# Autodesk Inventor assembly: Assembly1
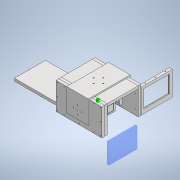
[picture p0: Inventor's stored thumbnail of the model, 180x180]
Saved by Autodesk Inventor 2022.2 (Build 262287030, 287C)
## iProperties
Created: 2022-01-28
Part Number: Assembly1
Document SubType Name: Assembly
Designer: Tapendra
Author: Tapendra
## Documents named in this file (25)
- C:\Users\Tapendra\Documents\opticalbox\Assembly1.iam
- C:\Users\Tapendra\Documents\opticalbox\base.ipt
- C:\Users\Tapendra\Documents\opticalbox\back.ipt
- C:\Users\Tapendra\Documents\opticalbox\top.ipt
- C:\Users\Tapendra\Documents\opticalbox\leftright.ipt
- C:\Users\Tapendra\Documents\opticalbox\CCM1-BS013.ipt
- C:\Users\Tapendra\Documents\opticalbox\front.ipt
- C:\Users\Tapendra\Documents\opticalbox\topwindow.ipt
- C:\Users\Tapendra\Documents\opticalbox\acrylicpmt.ipt
- C:\Users\Tapendra\Documents\opticalbox\toppmt.ipt
- C:\Users\Tapendra\Documents\opticalbox\left.ipt
- C:\Users\Tapendra\Documents\opticalbox\SM1D12-Step.ipt
- C:\Users\Tapendra\Documents\opticalbox\ELL14K-Step.ipt
- C:\Users\Tapendra\Documents\opticalbox\CFC11P-A-Step.ipt
- C:\Users\Tapendra\Documents\opticalbox\WP25M-UB-Step.ipt
- C:\Users\Tapendra\Documents\opticalbox\92078A216_Polycarbonate Dowel Pin.ipt
- C:\Users\Tapendra\Documents\opticalbox\baseblock.ipt
- C:\Users\Tapendra\Documents\opticalbox\baseplate.ipt
- C:\Users\Tapendra\Documents\opticalbox\MOT1102_0_3D.iam
- C:\Users\Tapendra\Documents\opticalbox\94180A351_Tapered Heat-Set Inserts for Plastic.ipt
- C:\Users\Tapendra\Documents\opticalbox\sidebracket.ipt
- C:\Users\Tapendra\Documents\opticalbox\pmtholder.ipt
- C:\Users\Tapendra\Documents\opticalbox\pmtbase.ipt
- C:\Users\Tapendra\Documents\Inventor\Content Center Files\R2022\en-US\UNI EN ISO 7045  H\EN ISO 7045 - M2 x  6 - 4.8 - H.ipt
- C:\Users\Tapendra\Documents\opticalbox\acrylicwindow.ipt
## Components (76 placed, 24 different names)
1. base:1 — Mate:1, Flush:1, Flush:2, Flush:8, Flush:9, Mate:15, Mate:24, Mate:25, Mate:26, Mate:27, Mate:33, Mate:34, Mate:35, Mate:57, Mate:60, Mate:61, Mate:64, Mate:86, Mate:92, Mate:131, Mate:132, Mate:133, Mate:134, Mate:135, Mate:136, Mate:137, Mate:138, Mate:144, Mate:145, Mate:146, Mate:147, Mate:148, Mate:149, Mate:150, Mate:151, Mate:153, Mate:154
2. back:1 — Mate:1, Flush:1, Flush:2, Mate:2, Flush:3, Flush:4, Mate:7, Mate:13, Mate:36, Mate:37, Mate:38, Mate:39, Mate:50, Mate:51, Mate:55, Mate:56, Mate:66, Mate:68, Mate:81, Mate:82, Mate:83, Mate:84, Mate:125, Mate:126, Mate:141, Mate:142
3. top:1 — Mate:2, Flush:3, Flush:4, Mate:5, Flush:6, Mate:6, Flush:7, Mate:73, Mate:74, Mate:75, Mate:76, Mate:77, Mate:78, Mate:79, Mate:80, Mate:94, Mate:95, Mate:96, Mate:97, Mate:98, Mate:99, Mate:100, Mate:101, Mate:102, Mate:103, Mate:104, Mate:105, Mate:106, Mate:107, Mate:108, Mate:109, Mate:110, Mate:111, Mate:112, Mate:113, Mate:114, Mate:115, Mate:116, Mate:117
4. front:1 — Mate:5, Flush:6, Mate:40, Mate:41, Mate:42, Mate:43, Mate:44, Mate:45, Mate:46, Mate:47, Mate:48, Mate:52, Mate:53, Mate:54, Mate:69, Mate:70, Mate:71, Mate:72, Mate:143
5. topwindow:1 — Mate:6, Flush:7, Mate:127, Mate:128, Mate:129, Mate:130
6. acrylicpmt:1 — Mate:85
7. leftright:1 — Mate:7, Flush:8, Mate:85
8. toppmt:1 — Mate:139, Mate:140
9. left:1 — Mate:13, Flush:9, Mate:86, Mate:143
10. CFC11P-A-Step:1 — Mate:30
11. ELL14K-Step:1 — Insert:1, Mate:22, Mate:23, Mate:30
12. WP25M-UB-Step:1 — Insert:1
13. CCM1-BS013:2 — Mate:17, Mate:18, Mate:22, Mate:23, Mate:87, Mate:88, Mate:122, Mate:152
14. 92078A216_Polycarbonate Dowel Pin:1 — Mate:40, Mate:41
15. 92078A216_Polycarbonate Dowel Pin:2 — Mate:26, Mate:27
16. 92078A216_Polycarbonate Dowel Pin:3 — Mate:15, Mate:33
17. 92078A216_Polycarbonate Dowel Pin:4 — Mate:144, Mate:145
18. 92078A216_Polycarbonate Dowel Pin:5 — Mate:34, Mate:35
19. 92078A216_Polycarbonate Dowel Pin:6 — Mate:146, Mate:147
20. 92078A216_Polycarbonate Dowel Pin:7 — Mate:24, Mate:25
21. 92078A216_Polycarbonate Dowel Pin:8 — Mate:38, Mate:39
22. 92078A216_Polycarbonate Dowel Pin:9 — Mate:36, Mate:37
23. SM1D12-Step:1 — Mate:17, Mate:18, Mate:121
24. 92078A216_Polycarbonate Dowel Pin:10 — Mate:53, Mate:54
25. 92078A216_Polycarbonate Dowel Pin:12 — Mate:60, Mate:61
26. 92078A216_Polycarbonate Dowel Pin:13 — Mate:42, Mate:43
27. 92078A216_Polycarbonate Dowel Pin:14 — Mate:50, Mate:56
28. 92078A216_Polycarbonate Dowel Pin:15 — Mate:44, Mate:45
29. 92078A216_Polycarbonate Dowel Pin:16 — Mate:46, Mate:47
30. 92078A216_Polycarbonate Dowel Pin:17 — Mate:48, Mate:52
31. 92078A216_Polycarbonate Dowel Pin:18 — Mate:148, Mate:149
32. 92078A216_Polycarbonate Dowel Pin:19 — Mate:57, Mate:64
33. 92078A216_Polycarbonate Dowel Pin:20 — Mate:150, Mate:151
34. 92078A216_Polycarbonate Dowel Pin:21 — Mate:141, Mate:142
35. 92078A216_Polycarbonate Dowel Pin:22 — Mate:66, Mate:68
36. 92078A216_Polycarbonate Dowel Pin:25 — Mate:51, Mate:55
37. 92078A216_Polycarbonate Dowel Pin:26 — Mate:75, Mate:77
38. 92078A216_Polycarbonate Dowel Pin:27 — Mate:70, Mate:71
39. 92078A216_Polycarbonate Dowel Pin:28 — Mate:74, Mate:79
40. 92078A216_Polycarbonate Dowel Pin:29 — Mate:76, Mate:78
41. 92078A216_Polycarbonate Dowel Pin:30 — Mate:73, Mate:80
42. 92078A216_Polycarbonate Dowel Pin:31 — Mate:81, Mate:82
43. 92078A216_Polycarbonate Dowel Pin:32 — Mate:69, Mate:72
44. 92078A216_Polycarbonate Dowel Pin:36 — Mate:83, Mate:84
45. baseblock:1 — Flush:91, Mate:90, Mate:91, Mate:92, Mate:153, Mate:154
46. baseplate:1 — Mate:87, Mate:88, Mate:89, Mate:91
47. 92078A216_Polycarbonate Dowel Pin:37 — Mate:89, Flush:91, Mate:90
48. MOT1102_0_3D:1 [sub-assembly]
49. 94180A351_Tapered Heat-Set Inserts for Plastic:1 — Mate:134, Mate:135
50. 94180A351_Tapered Heat-Set Inserts for Plastic:2 — Mate:96, Mate:107
51. 94180A351_Tapered Heat-Set Inserts for Plastic:3 — Mate:100, Mate:109
52. 94180A351_Tapered Heat-Set Inserts for Plastic:4 — Mate:102, Mate:111
53. 94180A351_Tapered Heat-Set Inserts for Plastic:5 — Mate:130
54. 94180A351_Tapered Heat-Set Inserts for Plastic:6 — Mate:106, Mate:115
55. 94180A351_Tapered Heat-Set Inserts for Plastic:7 — Mate:99, Mate:116
56. 94180A351_Tapered Heat-Set Inserts for Plastic:8 — Mate:101, Mate:110
57. 94180A351_Tapered Heat-Set Inserts for Plastic:9 — Mate:94, Mate:95
58. 94180A351_Tapered Heat-Set Inserts for Plastic:10 — Mate:97, Mate:108
59. 94180A351_Tapered Heat-Set Inserts for Plastic:11 — Mate:127
60. 94180A351_Tapered Heat-Set Inserts for Plastic:12 — Mate:131, Mate:132
61. 94180A351_Tapered Heat-Set Inserts for Plastic:13 — Mate:98, Mate:117
62. 94180A351_Tapered Heat-Set Inserts for Plastic:14 — Mate:129
63. 94180A351_Tapered Heat-Set Inserts for Plastic:15 — Mate:104, Mate:113
64. 94180A351_Tapered Heat-Set Inserts for Plastic:16 — Mate:105, Mate:114
65. 94180A351_Tapered Heat-Set Inserts for Plastic:17 — Mate:133, Mate:136
66. 94180A351_Tapered Heat-Set Inserts for Plastic:18 — Mate:128
67. 94180A351_Tapered Heat-Set Inserts for Plastic:19 — Mate:103, Mate:112
68. sidebracket:1 — Mate:125, Mate:126
69. pmtholder:1 — Mate:123, Mate:124
70. pmtbase:1 — Mate:121, Mate:122, Mate:123, Mate:124, Mate:139, Mate:140, Mate:152, Insert:3, Mate:155, Insert:4, Mate:156
71. 94180A351_Tapered Heat-Set Inserts for Plastic:20 — Mate:137, Mate:138
72. UNI EN ISO 7045 H M2 x  6 - 4.8 - H:1 — Mate:155
73. UNI EN ISO 7045 H M2 x  6 - 4.8 - H:2 — Mate:156
74. UNI EN ISO 7045 H M2 x  6 - 4.8 - H:3 — Insert:4
75. UNI EN ISO 7045 H M2 x  6 - 4.8 - H:4 — Insert:3
76. acrylicwindow:1
## Relationships (141: Mate 129, Flush 9, Insert 3)
- Mate:1: base:1 ↔ back:1
- Flush:1: base:1 ↔ back:1
- Flush:2: base:1 ↔ back:1
- Mate:2: back:1 ↔ top:1
- Flush:3: back:1 ↔ top:1
- Flush:4: back:1 ↔ top:1
- Mate:5: top:1 ↔ front:1
- Flush:6: top:1 ↔ front:1
- Mate:6: top:1 ↔ topwindow:1
- Flush:7: top:1 ↔ topwindow:1
- Mate:7: back:1 ↔ leftright:1
- Flush:8: base:1 ↔ leftright:1
- Mate:13: back:1 ↔ left:1
- Flush:9: base:1 ↔ left:1
- Insert:1 (-10 mm): ELL14K-Step:1 ↔ WP25M-UB-Step:1
- Mate:15: base:1 ↔ 92078A216_Polycarbonate Dowel Pin:3
- Mate:17: CCM1-BS013:2 ↔ SM1D12-Step:1
- Mate:18: CCM1-BS013:2 ↔ SM1D12-Step:1
- Mate:22: ELL14K-Step:1 ↔ CCM1-BS013:2
- Mate:23: ELL14K-Step:1 ↔ CCM1-BS013:2
- Mate:24: base:1 ↔ 92078A216_Polycarbonate Dowel Pin:7
- Mate:25: base:1 ↔ 92078A216_Polycarbonate Dowel Pin:7
- Mate:26: base:1 ↔ 92078A216_Polycarbonate Dowel Pin:2
- Mate:27: base:1 ↔ 92078A216_Polycarbonate Dowel Pin:2
- Mate:30: CFC11P-A-Step:1 ↔ ELL14K-Step:1
- Mate:33: base:1 ↔ 92078A216_Polycarbonate Dowel Pin:3
- Mate:34: base:1 ↔ 92078A216_Polycarbonate Dowel Pin:5
- Mate:35: base:1 ↔ 92078A216_Polycarbonate Dowel Pin:5
- Mate:36: back:1 ↔ 92078A216_Polycarbonate Dowel Pin:9
- Mate:37: back:1 ↔ 92078A216_Polycarbonate Dowel Pin:9
- Mate:38: back:1 ↔ 92078A216_Polycarbonate Dowel Pin:8
- Mate:39: back:1 ↔ 92078A216_Polycarbonate Dowel Pin:8
- Mate:40: front:1 ↔ 92078A216_Polycarbonate Dowel Pin:1
- Mate:41: front:1 ↔ 92078A216_Polycarbonate Dowel Pin:1
- Mate:42: front:1 ↔ 92078A216_Polycarbonate Dowel Pin:13
- Mate:43: front:1 ↔ 92078A216_Polycarbonate Dowel Pin:13
- Mate:44: front:1 ↔ 92078A216_Polycarbonate Dowel Pin:15
- Mate:45: front:1 ↔ 92078A216_Polycarbonate Dowel Pin:15
- Mate:46: front:1 ↔ 92078A216_Polycarbonate Dowel Pin:16
- Mate:47: front:1 ↔ 92078A216_Polycarbonate Dowel Pin:16
- Mate:48: front:1 ↔ 92078A216_Polycarbonate Dowel Pin:17
- Mate:50: back:1 ↔ 92078A216_Polycarbonate Dowel Pin:14
- Mate:51: back:1 ↔ 92078A216_Polycarbonate Dowel Pin:25
- Mate:52: front:1 ↔ 92078A216_Polycarbonate Dowel Pin:17
- Mate:53: front:1 ↔ 92078A216_Polycarbonate Dowel Pin:10
- Mate:54: front:1 ↔ 92078A216_Polycarbonate Dowel Pin:10
- Mate:55: back:1 ↔ 92078A216_Polycarbonate Dowel Pin:25
- Mate:56: back:1 ↔ 92078A216_Polycarbonate Dowel Pin:14
- Mate:57: base:1 ↔ 92078A216_Polycarbonate Dowel Pin:19
- Mate:60: base:1 ↔ 92078A216_Polycarbonate Dowel Pin:12
- Mate:61: base:1 ↔ 92078A216_Polycarbonate Dowel Pin:12
- Mate:64: base:1 ↔ 92078A216_Polycarbonate Dowel Pin:19
- Mate:66: back:1 ↔ 92078A216_Polycarbonate Dowel Pin:22
- Mate:68: back:1 ↔ 92078A216_Polycarbonate Dowel Pin:22
- Mate:69: front:1 ↔ 92078A216_Polycarbonate Dowel Pin:32
- Mate:70: front:1 ↔ 92078A216_Polycarbonate Dowel Pin:27
- Mate:71: front:1 ↔ 92078A216_Polycarbonate Dowel Pin:27
- Mate:72: front:1 ↔ 92078A216_Polycarbonate Dowel Pin:32
- Mate:73: top:1 ↔ 92078A216_Polycarbonate Dowel Pin:30
- Mate:74: top:1 ↔ 92078A216_Polycarbonate Dowel Pin:28
- Mate:75: top:1 ↔ 92078A216_Polycarbonate Dowel Pin:26
- Mate:76: top:1 ↔ 92078A216_Polycarbonate Dowel Pin:29
- Mate:77: top:1 ↔ 92078A216_Polycarbonate Dowel Pin:26
- Mate:78: top:1 ↔ 92078A216_Polycarbonate Dowel Pin:29
- Mate:79: top:1 ↔ 92078A216_Polycarbonate Dowel Pin:28
- Mate:80: top:1 ↔ 92078A216_Polycarbonate Dowel Pin:30
- Mate:81: back:1 ↔ 92078A216_Polycarbonate Dowel Pin:31
- Mate:82: back:1 ↔ 92078A216_Polycarbonate Dowel Pin:31
- Mate:83: back:1 ↔ 92078A216_Polycarbonate Dowel Pin:36
- Mate:84: back:1 ↔ 92078A216_Polycarbonate Dowel Pin:36
- Mate:85: acrylicpmt:1 ↔ leftright:1
- Mate:86: base:1 ↔ left:1
- Mate:87: CCM1-BS013:2 ↔ baseplate:1
- Mate:88: CCM1-BS013:2 ↔ baseplate:1
- Mate:89: baseplate:1 ↔ 92078A216_Polycarbonate Dowel Pin:37
- Flush:91: baseblock:1 ↔ 92078A216_Polycarbonate Dowel Pin:37
- Mate:90: baseblock:1 ↔ 92078A216_Polycarbonate Dowel Pin:37
- Mate:91: baseblock:1 ↔ baseplate:1
- Mate:92: base:1 ↔ baseblock:1
- Mate:94: top:1 ↔ 94180A351_Tapered Heat-Set Inserts for Plastic:9
- Mate:95: top:1 ↔ 94180A351_Tapered Heat-Set Inserts for Plastic:9
- Mate:96: top:1 ↔ 94180A351_Tapered Heat-Set Inserts for Plastic:2
- Mate:97: top:1 ↔ 94180A351_Tapered Heat-Set Inserts for Plastic:10
- Mate:98: top:1 ↔ 94180A351_Tapered Heat-Set Inserts for Plastic:13
- Mate:99: top:1 ↔ 94180A351_Tapered Heat-Set Inserts for Plastic:7
- Mate:100: top:1 ↔ 94180A351_Tapered Heat-Set Inserts for Plastic:3
- Mate:101: top:1 ↔ 94180A351_Tapered Heat-Set Inserts for Plastic:8
- Mate:102: top:1 ↔ 94180A351_Tapered Heat-Set Inserts for Plastic:4
- Mate:103: top:1 ↔ 94180A351_Tapered Heat-Set Inserts for Plastic:19
- Mate:104: top:1 ↔ 94180A351_Tapered Heat-Set Inserts for Plastic:15
- Mate:105: top:1 ↔ 94180A351_Tapered Heat-Set Inserts for Plastic:16
- Mate:106: top:1 ↔ 94180A351_Tapered Heat-Set Inserts for Plastic:6
- Mate:107: top:1 ↔ 94180A351_Tapered Heat-Set Inserts for Plastic:2
- Mate:108: top:1 ↔ 94180A351_Tapered Heat-Set Inserts for Plastic:10
- Mate:109: top:1 ↔ 94180A351_Tapered Heat-Set Inserts for Plastic:3
- Mate:110: top:1 ↔ 94180A351_Tapered Heat-Set Inserts for Plastic:8
- Mate:111: top:1 ↔ 94180A351_Tapered Heat-Set Inserts for Plastic:4
- Mate:112: top:1 ↔ 94180A351_Tapered Heat-Set Inserts for Plastic:19
- Mate:113: top:1 ↔ 94180A351_Tapered Heat-Set Inserts for Plastic:15
- Mate:114: top:1 ↔ 94180A351_Tapered Heat-Set Inserts for Plastic:16
- Mate:115: top:1 ↔ 94180A351_Tapered Heat-Set Inserts for Plastic:6
- Mate:116: top:1 ↔ 94180A351_Tapered Heat-Set Inserts for Plastic:7
- Mate:117: top:1 ↔ 94180A351_Tapered Heat-Set Inserts for Plastic:13
- Mate:121: SM1D12-Step:1 ↔ pmtbase:1
- Mate:122: CCM1-BS013:2 ↔ pmtbase:1
- Mate:123: pmtholder:1 ↔ pmtbase:1
- Mate:124: pmtholder:1 ↔ pmtbase:1
- Mate:125: back:1 ↔ sidebracket:1
- Mate:126 (20 mm): back:1 ↔ sidebracket:1
- Mate:127: topwindow:1 ↔ 94180A351_Tapered Heat-Set Inserts for Plastic:11
- Mate:128: topwindow:1 ↔ 94180A351_Tapered Heat-Set Inserts for Plastic:18
- Mate:129: topwindow:1 ↔ 94180A351_Tapered Heat-Set Inserts for Plastic:14
- Mate:130: topwindow:1 ↔ 94180A351_Tapered Heat-Set Inserts for Plastic:5
- Mate:131: base:1 ↔ 94180A351_Tapered Heat-Set Inserts for Plastic:12
- Mate:132: base:1 ↔ 94180A351_Tapered Heat-Set Inserts for Plastic:12
- Mate:133: base:1 ↔ 94180A351_Tapered Heat-Set Inserts for Plastic:17
- Mate:134: base:1 ↔ 94180A351_Tapered Heat-Set Inserts for Plastic:1
- Mate:135: base:1 ↔ 94180A351_Tapered Heat-Set Inserts for Plastic:1
- Mate:136: base:1 ↔ 94180A351_Tapered Heat-Set Inserts for Plastic:17
- Mate:137: base:1 ↔ 94180A351_Tapered Heat-Set Inserts for Plastic:20
- Mate:138: base:1 ↔ 94180A351_Tapered Heat-Set Inserts for Plastic:20
- Mate:139: toppmt:1 ↔ pmtbase:1
- Mate:140: toppmt:1 ↔ pmtbase:1
- Mate:141: back:1 ↔ 92078A216_Polycarbonate Dowel Pin:21
- Mate:142: back:1 ↔ 92078A216_Polycarbonate Dowel Pin:21
- Mate:143: front:1 ↔ left:1
- Mate:144: base:1 ↔ 92078A216_Polycarbonate Dowel Pin:4
- Mate:145: base:1 ↔ 92078A216_Polycarbonate Dowel Pin:4
- Mate:146: base:1 ↔ 92078A216_Polycarbonate Dowel Pin:6
- Mate:147: base:1 ↔ 92078A216_Polycarbonate Dowel Pin:6
- Mate:148: base:1 ↔ 92078A216_Polycarbonate Dowel Pin:18
- Mate:149: base:1 ↔ 92078A216_Polycarbonate Dowel Pin:18
- Mate:150: base:1 ↔ 92078A216_Polycarbonate Dowel Pin:20
- Mate:151: base:1 ↔ 92078A216_Polycarbonate Dowel Pin:20
- Mate:152: CCM1-BS013:2 ↔ pmtbase:1
- Mate:153: base:1 ↔ baseblock:1
- Mate:154: base:1 ↔ baseblock:1
- Insert:3: pmtbase:1 ↔ UNI EN ISO 7045 H M2 x  6 - 4.8 - H:4
- Mate:155: pmtbase:1 ↔ UNI EN ISO 7045 H M2 x  6 - 4.8 - H:1
- Insert:4: pmtbase:1 ↔ UNI EN ISO 7045 H M2 x  6 - 4.8 - H:3
- Mate:156: pmtbase:1 ↔ UNI EN ISO 7045 H M2 x  6 - 4.8 - H:2
